# Autodesk Inventor assembly: Assembly1
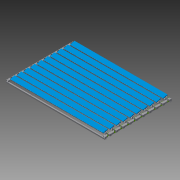
[picture p0: Inventor's stored thumbnail of the model, 180x180]
Saved by Autodesk Inventor 2015 SP1 (Build 190203100, 203)
## iProperties
Created: 2015-03-28
Part Number: Assembly1
Document SubType Name: Assembly
Designer: Cyril
Mass: 10678.5 g
Surface Area: 59183.2 cm^2
Volume: 10678.5 cm^3
Density: 1 g/cm^3
Author: Cyril
## Documents named in this file (12)
- C:\Users\Cyril\Documents\OSE FR\Concentrateur solaire\Inventor\Assemblage_cadre-miroir.iam
- C:\Users\Cyril\Documents\OSE FR\Concentrateur solaire\Inventor\Part4.ipt
- C:\Users\Cyril\Documents\OSE FR\Concentrateur solaire\Inventor\Assemblage_miroir.iam
- C:\Users\Cyril\Documents\OSE FR\Concentrateur solaire\Inventor\Moteur.ipt
- C:\Users\Cyril\Documents\OSE FR\Concentrateur solaire\Inventor\Accouplement.ipt
- C:\Users\Cyril\Documents\OSE FR\Concentrateur solaire\Inventor\michaud_chailly_C2_151_8_128.ipt
- C:\Users\Cyril\Documents\OSE FR\Concentrateur solaire\Inventor\Plaque support_D.ipt
- C:\Users\Cyril\Documents\OSE FR\Concentrateur solaire\Inventor\Assemblage_Cadre.iam
- C:\Users\Cyril\Documents\OSE FR\Concentrateur solaire\Inventor\Capteur optique.ipt
- C:\Users\Cyril\Documents\OSE FR\Concentrateur solaire\Inventor\Plaque support_G.ipt
- C:\Users\Cyril\Documents\OSE FR\Concentrateur solaire\Inventor\Bibliothèque\Imported Components\Hexagon_head_bolt_DINENISO4014_M6_55\Hexagon_head_bolt_DINENISO4014_M6_55.ipt
- C:\Users\Cyril\Documents\OSE FR\Concentrateur solaire\Imported Components\test export STEP\test export STEP.ipt
## Components (95 placed, 11 different names)
1. Assemblage_Cadre:1 [sub-assembly] — Insert:37, Flush:34, Flush:35, Flush:36, Insert:38, Insert:39, Insert:40, Insert:41, Insert:43
2. Hexagon_head_bolt_DINENISO4014_M6_55:2 — Insert:45
3. Hexagon_head_bolt_DINENISO4014_M6_55:3 — Insert:44
4. test export STEP:2 — Insert:48
5. test export STEP:3 — Insert:47
6. Moteur:1 — Insert:19, Insert:23, Insert:24
7. Part4:1 — Insert:23, Insert:24, Insert:37, Insert:38, Insert:47, Insert:48
8. Plaque support_D:1 — Insert:21, Insert:25, Mate:4, Insert:39, Insert:43, Insert:44, Insert:45
9. Assemblage_miroir:3 [sub-assembly] — Insert:20, Mate:3
10. michaud_chailly_C2_151_8_128:1 — Insert:21, Mate:3
11. Accouplement:1 — Insert:19, Insert:20
12. Capteur optique:1 — Insert:25, Mate:4
13. Plaque support_G:1 — Insert:40, Insert:41, Insert:42
14. michaud_chailly_C2_151_8_128:11 — Insert:42
15. Moteur:2
16. Part4:2
17. Plaque support_D:3
18. Assemblage_miroir:4 [sub-assembly]
19. michaud_chailly_C2_151_8_128:2
20. Accouplement:2
21. Capteur optique:2
22. Plaque support_G:2
23. michaud_chailly_C2_151_8_128:12
24. Moteur:3
25. Part4:3
26. Plaque support_D:4
27. Assemblage_miroir:5 [sub-assembly]
28. michaud_chailly_C2_151_8_128:3
29. Accouplement:3
30. Capteur optique:3
31. Plaque support_G:3
32. michaud_chailly_C2_151_8_128:13
33. Moteur:4
34. Part4:4
35. Plaque support_D:5
36. Assemblage_miroir:6 [sub-assembly]
37. michaud_chailly_C2_151_8_128:4
38. Accouplement:4
39. Capteur optique:4
40. Plaque support_G:4
41. michaud_chailly_C2_151_8_128:14
42. Moteur:5
43. Part4:5
44. Plaque support_D:6
45. Assemblage_miroir:7 [sub-assembly]
46. michaud_chailly_C2_151_8_128:5
47. Accouplement:5
48. Capteur optique:5
49. Plaque support_G:5
50. michaud_chailly_C2_151_8_128:15
51. Moteur:6
52. Part4:6
53. Plaque support_D:7
54. Assemblage_miroir:8 [sub-assembly]
55. michaud_chailly_C2_151_8_128:6
56. Accouplement:6
57. Capteur optique:6
58. Plaque support_G:6
59. michaud_chailly_C2_151_8_128:16
60. Moteur:7
61. Part4:7
62. Plaque support_D:8
63. Assemblage_miroir:9 [sub-assembly]
64. michaud_chailly_C2_151_8_128:7
65. Accouplement:7
66. Capteur optique:7
67. Plaque support_G:7
68. michaud_chailly_C2_151_8_128:17
69. Moteur:8
70. Part4:8
71. Plaque support_D:9
72. Assemblage_miroir:10 [sub-assembly]
73. michaud_chailly_C2_151_8_128:8
74. Accouplement:8
75. Capteur optique:8
76. Plaque support_G:8
77. michaud_chailly_C2_151_8_128:18
78. Moteur:9
79. Part4:9
80. Plaque support_D:10
81. Assemblage_miroir:11 [sub-assembly]
82. michaud_chailly_C2_151_8_128:9
83. Accouplement:9
84. Capteur optique:9
85. Plaque support_G:9
86. michaud_chailly_C2_151_8_128:19
87. Moteur:10
88. Part4:10
89. Plaque support_D:11
90. Assemblage_miroir:12 [sub-assembly]
91. michaud_chailly_C2_151_8_128:10
92. Accouplement:10
93. Capteur optique:10
94. Plaque support_G:10
95. michaud_chailly_C2_151_8_128:20
## Component patterns: (10 elements, first: Moteur:1 + Part4:1 + Plaque support_D:1 + Assemblage_miroir:3 + michaud_chailly_C2_151_8_128:1 + Accouplement:1 + Capteur optique:1 + Plaque support_G:1 + michaud_chailly_C2_151_8_128:11)
## Relationships (22: Insert 17, Flush 3, Mate 2)
- Insert:19 (-10 mm): Moteur:1 ↔ Accouplement:1
- Insert:20 (-8 mm): Assemblage_miroir:3 ↔ Accouplement:1
- Insert:21: Plaque support_D:1 ↔ michaud_chailly_C2_151_8_128:1
- Insert:23: Moteur:1 ↔ Part4:1
- Insert:24: Moteur:1 ↔ Part4:1
- Mate:3: Assemblage_miroir:3 ↔ michaud_chailly_C2_151_8_128:1
- Insert:25: Plaque support_D:1 ↔ Capteur optique:1
- Mate:4: Plaque support_D:1 ↔ Capteur optique:1
- Insert:37: Assemblage_Cadre:1 ↔ Part4:1
- Flush:34: Assemblage_Cadre:1
- Flush:35: Assemblage_Cadre:1
- Flush:36: Assemblage_Cadre:1
- Insert:38: Assemblage_Cadre:1 ↔ Part4:1
- Insert:39: Assemblage_Cadre:1 ↔ Plaque support_D:1
- Insert:40: Assemblage_Cadre:1 ↔ Plaque support_G:1
- Insert:41: Assemblage_Cadre:1 ↔ Plaque support_G:1
- Insert:42: Plaque support_G:1 ↔ michaud_chailly_C2_151_8_128:11
- Insert:43: Assemblage_Cadre:1 ↔ Plaque support_D:1
- Insert:44: Hexagon_head_bolt_DINENISO4014_M6_55:3 ↔ Plaque support_D:1
- Insert:45: Hexagon_head_bolt_DINENISO4014_M6_55:2 ↔ Plaque support_D:1
- Insert:47: test export STEP:3 ↔ Part4:1
- Insert:48: test export STEP:2 ↔ Part4:1
